# Autodesk Inventor assembly: Main_Station
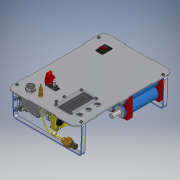
[picture p0: Inventor's stored thumbnail of the model, 180x180]
Saved by Autodesk Inventor 2016 (Build 200138000, 138)
## iProperties
Created: 2016-03-26
Part Number: Main_Station
Document SubType Name: Assembly
Designer: agmle
Author: agmle
## Documents named in this file (42)
- C:\Users\agmle\BitTorrent Sync\private\projects\Creekfleet_Timer\hardware\CAD\Main\Main_Station.iam
- C:\Users\agmle\BitTorrent Sync\private\projects\Creekfleet_Timer\hardware\CAD\Main\Case.ipt
- C:\Users\agmle\BitTorrent Sync\private\projects\Creekfleet_Timer\hardware\CAD\Main\Panel_Strut.ipt
- C:\Users\agmle\BitTorrent Sync\private\projects\Creekfleet_Timer\hardware\CAD\Main\VIAIR 90Cviair_90c_compressor_avp.ipt
- C:\Users\agmle\BitTorrent Sync\private\projects\Creekfleet_Timer\hardware\CAD\Main\Compressor_Strut.ipt
- C:\Users\agmle\BitTorrent Sync\private\projects\Creekfleet_Timer\hardware\CAD\Main\Panel.ipt
- C:\Users\agmle\BitTorrent Sync\private\projects\Creekfleet_Timer\hardware\CAD\Main\RKF 46-1M_NPT.ipt
- C:\Users\agmle\Documents\Inventor\Content Center Files\R2016\en-US\ANSI B18.22.1\ANSI B18.22.1 - No. 4 - Regular - Type B.ipt
- C:\Users\agmle\Documents\Inventor\Content Center Files\R2016\en-US\ANSI B18.22.1\ANSI B18.22.1 - 1_4 - narrow - Type B.ipt
- C:\Users\agmle\Documents\Inventor\Content Center Files\R2016\en-US\ASME B18.21.1(08)\ASME B18.21.1 - No. 4. Carbon Steel(2) A.ipt
- C:\Users\agmle\Documents\Inventor\Content Center Files\R2016\en-US\ASME B18.21.1(08)\ASME B18.21.1 - 1_4. Carbon Steel(2) A.ipt
- C:\Users\agmle\Documents\Inventor\Content Center Files\R2016\en-US\ANSI B18.3(03)\ANSI B18.3 - 1_4-20 UNC - UNC - 0.625(1).ipt
- C:\Users\agmle\Documents\Inventor\Content Center Files\R2016\en-US\ANSI B18.3(05)\ANSI B18.3 - 4-40 UNC - 0.3125(31).ipt
- C:\Users\agmle\BitTorrent Sync\private\projects\Creekfleet_Timer\hardware\CAD\Main\LCD.iam
- C:\Users\agmle\BitTorrent Sync\private\projects\Creekfleet_Timer\hardware\CAD\Main\LCD_Cover.ipt
- C:\Users\agmle\Documents\Inventor\Content Center Files\R2016\en-US\ANSI B18.3(05)\ANSI B18.3 - 4-40 UNC - 0.875(31).ipt
- C:\Users\agmle\Documents\Inventor\Content Center Files\R2016\en-US\ANSI B18.6.3(36)\ANSI B18.6.3 - 4 - 40(2).ipt
- C:\Users\agmle\BitTorrent Sync\private\projects\Creekfleet_Timer\hardware\CAD\Main\toggle switch cover.iam
- C:\Users\agmle\BitTorrent Sync\private\projects\Creekfleet_Timer\hardware\CAD\Main\Button_blue.iam
- C:\Users\agmle\BitTorrent Sync\private\projects\Creekfleet_Timer\hardware\CAD\Main\Button_green.iam
- C:\Users\agmle\BitTorrent Sync\private\projects\Creekfleet_Timer\hardware\CAD\Main\Button_red.iam
- C:\Users\agmle\BitTorrent Sync\private\projects\Creekfleet_Timer\hardware\CAD\Main\9414K930.ipt
- C:\Users\agmle\BitTorrent Sync\private\projects\Creekfleet_Timer\hardware\CAD\Main\9414K360.ipt
- C:\Users\agmle\BitTorrent Sync\private\projects\Creekfleet_Timer\hardware\CAD\Main\5454K650.ipt
- C:\Users\agmle\BitTorrent Sync\private\projects\Creekfleet_Timer\hardware\CAD\Main\50745K260.ipt
- C:\Users\agmle\BitTorrent Sync\private\projects\Creekfleet_Timer\hardware\CAD\Main\PX3AN2BS250PAAAX.ipt
- C:\Users\agmle\BitTorrent Sync\private\projects\Creekfleet_Timer\hardware\CAD\Main\2844K430.ipt
- C:\Users\agmle\BitTorrent Sync\private\projects\Creekfleet_Timer\hardware\CAD\Main\Main_Station\AIP\Tube and Pipe\Main_Station.Airline.iam
- C:\Users\agmle\BitTorrent Sync\private\projects\Creekfleet_Timer\hardware\CAD\Main\Toggle_Switch.iam
- C:\Users\agmle\BitTorrent Sync\private\projects\Creekfleet_Timer\hardware\CAD\Main\Toggle_Nut.ipt
- C:\Users\agmle\BitTorrent Sync\private\projects\Creekfleet_Timer\hardware\CAD\Main\BMS.ipt
- C:\Users\agmle\BitTorrent Sync\private\projects\Creekfleet_Timer\hardware\CAD\Main\40152S.ipt
- C:\Users\agmle\BitTorrent Sync\private\projects\Creekfleet_Timer\hardware\CAD\Main\Cell_Spacer.ipt
- C:\Users\agmle\BitTorrent Sync\private\projects\Creekfleet_Timer\hardware\CAD\Main\black_pp45.ipt
- C:\Users\agmle\BitTorrent Sync\private\projects\Creekfleet_Timer\hardware\CAD\Main\red_pp45.ipt
- C:\Users\agmle\BitTorrent Sync\private\projects\Creekfleet_Timer\hardware\CAD\Main\1470g1.ipt
- C:\Users\agmle\BitTorrent Sync\private\projects\Creekfleet_Timer\hardware\CAD\Main\AFB0512HA.ipt
- C:\Users\agmle\BitTorrent Sync\private\projects\Creekfleet_Timer\hardware\CAD\Main\Fan_Bracket.ipt
- C:\Users\agmle\Documents\Inventor\Content Center Files\R2016\en-US\ANSI B18.22.1\ANSI B18.22.1 - No. 8 - narrow - Type B.ipt
- C:\Users\agmle\Documents\Inventor\Content Center Files\R2016\en-US\ANSI B18.6.3(36)\ANSI B18.6.3 - 10 - 32(2).ipt
- C:\Users\agmle\Documents\Inventor\Content Center Files\R2016\en-US\ANSI B18.3(05)\ANSI B18.3 - 8-36 UNF - 0.875(31).ipt
- C:\Users\agmle\Documents\Inventor\Content Center Files\R2016\en-US\ASME B18.21.1(08)\ASME B18.21.1 - No. 8. Carbon Steel(2) A.ipt
## Components (123 placed, 41 different names)
1. Case:1 — Mate:1, Mate:2, Mate:3, Mate:4, Mate:5, Mate:6, Mate:7, Mate:8, Angle:2, Angle:3
2. Panel_Strut:1 — Mate:1, Mate:2, Mate:6, Insert:17, Insert:20, Insert:21, Mate:36, Mate:37, Mate:38, Angle:6
3. Panel_Strut:2 — Mate:3, Mate:4, Mate:5, Insert:14, Insert:16, Insert:22, Flush:2, Mate:35
4. VIAIR 90Cviair_90c_compressor_avp:1 — Insert:23, Insert:24, Insert:54, Insert:55, Insert:56, Insert:57, Insert:100
5. Compressor_Strut:1 — Insert:14, Insert:20, Insert:24, Insert:50, Insert:52, Mate:16
6. Compressor_Strut:2 — Insert:16, Insert:17, Insert:23, Insert:51, Insert:53
7. Panel:1 — Insert:21, Insert:22, Insert:25, Insert:46, Insert:47, Insert:48, Flush:1, Insert:74, Insert:87, Insert:88, Insert:94, Insert:95, Insert:96, Insert:97, Insert:98, Insert:102, Angle:5, Mate:17, Mate:34, Mate:41, Mate:42, Mate:43, Insert:125, Mate:49, Insert:130, Insert:131
8. RKF 46-1M_NPT:1 — Insert:25
9. Plain Washer (Inch) No. 4 - Regular - Type B:1 — Insert:30, Insert:46
10. Plain Washer (Inch) No. 4 - Regular - Type B:2 — Insert:31, Insert:47
11. Plain Washer (Inch) No. 4 - Regular - Type B:3 — Insert:32, Insert:48
12. Plain Washer (Inch) No. 4 - Regular - Type B:5 — Insert:34, Insert:50
13. Plain Washer (Inch) No. 4 - Regular - Type B:6 — Insert:35, Insert:51
14. Plain Washer (Inch) No. 4 - Regular - Type B:7 — Insert:36, Insert:52
15. Plain Washer (Inch) No. 4 - Regular - Type B:8 — Insert:37, Insert:53
16. Plain Washer (Inch) 1/4 - narrow - Type B:1 — Insert:29, Insert:56
17. Plain Washer (Inch) 1/4 - narrow - Type B:2 — Insert:28, Insert:57
18. Plain Washer (Inch) 1/4 - narrow - Type B:3 — Insert:27, Insert:55
19. Plain Washer (Inch) 1/4 - narrow - Type B:4 — Insert:26, Insert:54
20. Internal Tooth Lock Washer - Type A (Inch) No. 4. Carbon Steel:1 — Insert:30, Insert:45
21. Internal Tooth Lock Washer - Type A (Inch) No. 4. Carbon Steel:2 — Insert:31, Insert:44
22. Internal Tooth Lock Washer - Type A (Inch) No. 4. Carbon Steel:3 — Insert:32, Insert:43
23. Internal Tooth Lock Washer - Type A (Inch) No. 4. Carbon Steel:5 — Insert:34, Insert:41
24. Internal Tooth Lock Washer - Type A (Inch) No. 4. Carbon Steel:6 — Insert:35, Insert:40
25. Internal Tooth Lock Washer - Type A (Inch) No. 4. Carbon Steel:7 — Insert:36, Insert:39
26. Internal Tooth Lock Washer - Type A (Inch) No. 4. Carbon Steel:8 — Insert:37, Insert:38
27. Internal Tooth Lock Washer - Type A (Inch) 1/4. Carbon Steel:1 — Insert:26
28. Internal Tooth Lock Washer - Type A (Inch) 1/4. Carbon Steel:2 — Insert:27
29. Internal Tooth Lock Washer - Type A (Inch) 1/4. Carbon Steel:3 — Insert:28
30. Internal Tooth Lock Washer - Type A (Inch) 1/4. Carbon Steel:4 — Insert:29
31. Hexagon Socket Head Cap Screw - Inch No. 4 - 40 UNC - 5/16:2 — Insert:45
32. Hexagon Socket Head Cap Screw - Inch No. 4 - 40 UNC - 5/16:3 — Insert:44
33. Hexagon Socket Head Cap Screw - Inch No. 4 - 40 UNC - 5/16:4 — Insert:43
34. Hexagon Socket Head Cap Screw - Inch No. 4 - 40 UNC - 5/16:6 — Insert:41
35. Hexagon Socket Head Cap Screw - Inch No. 4 - 40 UNC - 5/16:7 — Insert:40
36. Hexagon Socket Head Cap Screw - Inch No. 4 - 40 UNC - 5/16:1 — Insert:39
37. Hexagon Socket Head Cap Screw - Inch No. 4 - 40 UNC - 5/16:8 — Insert:38
38. Hexagon Socket Button Head Cap Screw - Inch 1/4 - 20 x 5/8:1
39. Hexagon Socket Button Head Cap Screw - Inch 1/4 - 20 x 5/8:2
40. Hexagon Socket Button Head Cap Screw - Inch 1/4 - 20 x 5/8:3
41. Hexagon Socket Button Head Cap Screw - Inch 1/4 - 20 x 5/8:4
42. LCD:1 [sub-assembly] — Flush:1, Mate:9, Mate:10, Insert:79, Insert:80, Insert:81, Insert:82
43. LCD_Cover:1 — Insert:87, Insert:88, Insert:89, Insert:90, Insert:91, Insert:92
44. Plain Washer (Inch) No. 4 - Regular - Type B:9 — Insert:64, Insert:74
45. Plain Washer (Inch) No. 4 - Regular - Type B:10 — Insert:65, Insert:89
46. Plain Washer (Inch) No. 4 - Regular - Type B:11 — Insert:66, Insert:90
47. Plain Washer (Inch) No. 4 - Regular - Type B:12 — Insert:67, Insert:91
48. Plain Washer (Inch) No. 4 - Regular - Type B:13 — Insert:68, Insert:92
49. Internal Tooth Lock Washer - Type A (Inch) No. 4. Carbon Steel:9 — Insert:64, Insert:69
50. Internal Tooth Lock Washer - Type A (Inch) No. 4. Carbon Steel:10 — Insert:65, Insert:70
51. Internal Tooth Lock Washer - Type A (Inch) No. 4. Carbon Steel:11 — Insert:66, Insert:71
52. Internal Tooth Lock Washer - Type A (Inch) No. 4. Carbon Steel:12 — Insert:67, Insert:72
53. Internal Tooth Lock Washer - Type A (Inch) No. 4. Carbon Steel:13 — Insert:68, Insert:73
54. Hexagon Socket Head Cap Screw - Inch No. 4 - 40 UNC - 5/16:9 — Insert:69
55. Hexagon Socket Head Cap Screw - Inch No. 4 - 40 UNC - 7/8:2 — Insert:70, Mate:9
56. Hexagon Socket Head Cap Screw - Inch No. 4 - 40 UNC - 7/8:1 — Insert:71
57. Hexagon Socket Head Cap Screw - Inch No. 4 - 40 UNC - 7/8:3 — Insert:72, Mate:10
58. Hexagon Socket Head Cap Screw - Inch No. 4 - 40 UNC - 7/8:4 — Insert:73
59. Hex Machine Screw Nut - Inch 4 - 40:1 — Insert:79, Insert:86
60. Hex Machine Screw Nut - Inch 4 - 40:2 — Insert:80, Insert:83
61. Hex Machine Screw Nut - Inch 4 - 40:3 — Insert:81, Insert:85
62. Hex Machine Screw Nut - Inch 4 - 40:4 — Insert:82, Insert:84
63. Hex Machine Screw Nut - Inch 4 - 40:5 — Insert:84
64. Hex Machine Screw Nut - Inch 4 - 40:6 — Insert:83
65. Hex Machine Screw Nut - Inch 4 - 40:7 — Insert:86
66. Hex Machine Screw Nut - Inch 4 - 40:8 — Insert:85
67. toggle switch cover:1 [sub-assembly] — Insert:94, Angle:3, Insert:103
68. Button_red:1 [sub-assembly] — Insert:95
69. Button_blue:1 [sub-assembly] — Insert:97
70. Button_green:1 [sub-assembly] — Insert:96
71. 9414K930:1 — Insert:98, Angle:2, Insert:99
72. 9414K360:1 — Insert:99
73. 5454K650:1 — Insert:100
74. 50745K260:1 — Insert:101, Mate:38, Mate:39, Mate:40
75. PX3AN2BS250PAAAX:1 — Insert:101, Mate:36, Mate:37
76. 2844K430:1 — Mate:39, Angle:6, Mate:40
77. Main_Station.Airline:1 [sub-assembly]
78. Toggle_Switch:1 [sub-assembly] — Insert:102, Angle:5
79. Toggle_Nut:1 — Insert:103
80. BMS:1 — Mate:16, Flush:2, Mate:17, Flush:12
81. 40152S:1 — Mate:18, Mate:19, Flush:3
82. 40152S:2 — Mate:20, Mate:21, Flush:9
83. 40152S:3 — Mate:22, Mate:23, Flush:8, Flush:9
84. 40152S:4 — Mate:24, Mate:25, Flush:3, Flush:4
85. 40152S:5 — Mate:26, Mate:27, Flush:7, Flush:8
86. 40152S:6 — Mate:32, Mate:33, Flush:5, Flush:6, Flush:10, Flush:11
87. 40152S:7 — Mate:28, Mate:29, Flush:6, Flush:7
88. 40152S:8 — Mate:30, Mate:31, Flush:4, Flush:5
89. Cell_Spacer:1 — Mate:18, Mate:20, Mate:22, Mate:24, Mate:26, Mate:28, Mate:30, Mate:32, Flush:10, Mate:34, Flush:12, Mate:35
90. Cell_Spacer:2 — Mate:19, Mate:21, Mate:23, Mate:25, Mate:27, Mate:29, Mate:31, Mate:33, Flush:11
91. black_pp45:1 — Flush:13, Mate:44, Mate:47, Flush:16
92. black_pp45:2 — Flush:15, Mate:45, Mate:47, Flush:16, Flush:18, Flush:20
93. red_pp45:1 — Flush:13, Flush:14, Mate:44, Mate:46, Flush:17
94. red_pp45:2 — Flush:14, Flush:15, Mate:45, Mate:46, Flush:18, Flush:19
95. 1470g1:2 — Mate:41, Mate:42, Mate:43, Flush:17, Flush:19, Flush:20
96. AFB0512HA:1 — Insert:104, Mate:48, Insert:121, Insert:122, Insert:123, Insert:124
97. Fan_Bracket:1 — Insert:104, Mate:48, Insert:117, Insert:118, Insert:119, Insert:120, Insert:125, Mate:49
98. Hexagon Socket Head Cap Screw - Inch 8-36 UNF - 0.875:2 — Insert:105
99. Plain Washer (Inch) No. 8 - narrow - Type B:1 — Insert:105, Insert:117
100. Plain Washer (Inch) No. 8 - narrow - Type B:2 — Insert:121
101. Internal Tooth Lock Washer - Type A (Inch) No. 8. Carbon Steel:4
102. Hex Machine Screw Nut - Inch 10 - 32:1
103. Hexagon Socket Head Cap Screw - Inch 8-36 UNF - 0.875:3
104. Plain Washer (Inch) No. 8 - narrow - Type B:3 — Insert:119
105. Plain Washer (Inch) No. 8 - narrow - Type B:4 — Insert:124
106. Internal Tooth Lock Washer - Type A (Inch) No. 8. Carbon Steel:3
107. Hex Machine Screw Nut - Inch 10 - 32:2
108. Hexagon Socket Head Cap Screw - Inch 8-36 UNF - 0.875:4
109. Plain Washer (Inch) No. 8 - narrow - Type B:5 — Insert:120
110. Plain Washer (Inch) No. 8 - narrow - Type B:6 — Insert:123
111. Internal Tooth Lock Washer - Type A (Inch) No. 8. Carbon Steel:2
112. Hex Machine Screw Nut - Inch 10 - 32:3
113. Hexagon Socket Head Cap Screw - Inch 8-36 UNF - 0.875:1
114. Plain Washer (Inch) No. 8 - narrow - Type B:7 — Insert:118
115. Plain Washer (Inch) No. 8 - narrow - Type B:8 — Insert:122
116. Internal Tooth Lock Washer - Type A (Inch) No. 8. Carbon Steel:1
117. Hex Machine Screw Nut - Inch 10 - 32:4
118. Plain Washer (Inch) No. 4 - Regular - Type B:14 — Insert:130
119. Internal Tooth Lock Washer - Type A (Inch) No. 4. Carbon Steel:14
120. Hexagon Socket Head Cap Screw - Inch No. 4 - 40 UNC - 7/8:5
121. Plain Washer (Inch) No. 4 - Regular - Type B:15 — Insert:131
122. Internal Tooth Lock Washer - Type A (Inch) No. 4. Carbon Steel:15
123. Hexagon Socket Head Cap Screw - Inch No. 4 - 40 UNC - 7/8:6
## Relationships (173: Insert 105, Mate 44, Flush 20, Angle 4)
- Mate:1: Case:1 ↔ Panel_Strut:1
- Mate:2: Case:1 ↔ Panel_Strut:1
- Mate:3: Case:1 ↔ Panel_Strut:2
- Mate:4: Case:1 ↔ Panel_Strut:2
- Mate:5: Case:1 ↔ Panel_Strut:2
- Mate:6: Case:1 ↔ Panel_Strut:1
- Insert:14: Panel_Strut:2 ↔ Compressor_Strut:1
- Insert:16: Panel_Strut:2 ↔ Compressor_Strut:2
- Insert:17: Panel_Strut:1 ↔ Compressor_Strut:2
- Insert:20: Panel_Strut:1 ↔ Compressor_Strut:1
- Insert:21: Panel_Strut:1 ↔ Panel:1
- Insert:22: Panel_Strut:2 ↔ Panel:1
- Insert:23: VIAIR 90Cviair_90c_compressor_avp:1 ↔ Compressor_Strut:2
- Insert:24: VIAIR 90Cviair_90c_compressor_avp:1 ↔ Compressor_Strut:1
- Insert:25: Panel:1 ↔ RKF 46-1M_NPT:1
- Insert:26: Plain Washer (Inch) 1/4 - narrow - Type B:4 ↔ Internal Tooth Lock Washer - Type A (Inch) 1/4. Carbon Steel:1
- Insert:27: Plain Washer (Inch) 1/4 - narrow - Type B:3 ↔ Internal Tooth Lock Washer - Type A (Inch) 1/4. Carbon Steel:2
- Insert:28: Plain Washer (Inch) 1/4 - narrow - Type B:2 ↔ Internal Tooth Lock Washer - Type A (Inch) 1/4. Carbon Steel:3
- Insert:29: Plain Washer (Inch) 1/4 - narrow - Type B:1 ↔ Internal Tooth Lock Washer - Type A (Inch) 1/4. Carbon Steel:4
- Insert:30: Plain Washer (Inch) No. 4 - Regular - Type B:1 ↔ Internal Tooth Lock Washer - Type A (Inch) No. 4. Carbon Steel:1
- Insert:31: Plain Washer (Inch) No. 4 - Regular - Type B:2 ↔ Internal Tooth Lock Washer - Type A (Inch) No. 4. Carbon Steel:2
- Insert:32: Plain Washer (Inch) No. 4 - Regular - Type B:3 ↔ Internal Tooth Lock Washer - Type A (Inch) No. 4. Carbon Steel:3
- Insert:34: Plain Washer (Inch) No. 4 - Regular - Type B:5 ↔ Internal Tooth Lock Washer - Type A (Inch) No. 4. Carbon Steel:5
- Insert:35: Plain Washer (Inch) No. 4 - Regular - Type B:6 ↔ Internal Tooth Lock Washer - Type A (Inch) No. 4. Carbon Steel:6
- Insert:36: Plain Washer (Inch) No. 4 - Regular - Type B:7 ↔ Internal Tooth Lock Washer - Type A (Inch) No. 4. Carbon Steel:7
- Insert:37: Plain Washer (Inch) No. 4 - Regular - Type B:8 ↔ Internal Tooth Lock Washer - Type A (Inch) No. 4. Carbon Steel:8
- Insert:38: Internal Tooth Lock Washer - Type A (Inch) No. 4. Carbon Steel:8 ↔ Hexagon Socket Head Cap Screw - Inch No. 4 - 40 UNC - 5/16:8
- Insert:39: Internal Tooth Lock Washer - Type A (Inch) No. 4. Carbon Steel:7 ↔ Hexagon Socket Head Cap Screw - Inch No. 4 - 40 UNC - 5/16:1
- Insert:40: Internal Tooth Lock Washer - Type A (Inch) No. 4. Carbon Steel:6 ↔ Hexagon Socket Head Cap Screw - Inch No. 4 - 40 UNC - 5/16:7
- Insert:41: Internal Tooth Lock Washer - Type A (Inch) No. 4. Carbon Steel:5 ↔ Hexagon Socket Head Cap Screw - Inch No. 4 - 40 UNC - 5/16:6
- Insert:43: Internal Tooth Lock Washer - Type A (Inch) No. 4. Carbon Steel:3 ↔ Hexagon Socket Head Cap Screw - Inch No. 4 - 40 UNC - 5/16:4
- Insert:44: Internal Tooth Lock Washer - Type A (Inch) No. 4. Carbon Steel:2 ↔ Hexagon Socket Head Cap Screw - Inch No. 4 - 40 UNC - 5/16:3
- Insert:45: Internal Tooth Lock Washer - Type A (Inch) No. 4. Carbon Steel:1 ↔ Hexagon Socket Head Cap Screw - Inch No. 4 - 40 UNC - 5/16:2
- Insert:46: Panel:1 ↔ Plain Washer (Inch) No. 4 - Regular - Type B:1
- Insert:47: Panel:1 ↔ Plain Washer (Inch) No. 4 - Regular - Type B:2
- Insert:48: Panel:1 ↔ Plain Washer (Inch) No. 4 - Regular - Type B:3
- Insert:50: Compressor_Strut:1 ↔ Plain Washer (Inch) No. 4 - Regular - Type B:5
- Insert:51: Compressor_Strut:2 ↔ Plain Washer (Inch) No. 4 - Regular - Type B:6
- Insert:52: Compressor_Strut:1 ↔ Plain Washer (Inch) No. 4 - Regular - Type B:7
- Insert:53: Compressor_Strut:2 ↔ Plain Washer (Inch) No. 4 - Regular - Type B:8
- Insert:54: VIAIR 90Cviair_90c_compressor_avp:1 ↔ Plain Washer (Inch) 1/4 - narrow - Type B:4
- Insert:55: VIAIR 90Cviair_90c_compressor_avp:1 ↔ Plain Washer (Inch) 1/4 - narrow - Type B:3
- Insert:56: VIAIR 90Cviair_90c_compressor_avp:1 ↔ Plain Washer (Inch) 1/4 - narrow - Type B:1
- Insert:57: VIAIR 90Cviair_90c_compressor_avp:1 ↔ Plain Washer (Inch) 1/4 - narrow - Type B:2
- [Insert]: Internal Tooth Lock Washer - Type A (Inch) 1/4. Carbon Steel:4 ↔ Hexagon Socket Button Head Cap Screw - Inch 1/4 - 20 x 5/8:1
- [Insert]: Internal Tooth Lock Washer - Type A (Inch) 1/4. Carbon Steel:3 ↔ Hexagon Socket Button Head Cap Screw - Inch 1/4 - 20 x 5/8:2
- [Insert]: Internal Tooth Lock Washer - Type A (Inch) 1/4. Carbon Steel:1 ↔ Hexagon Socket Button Head Cap Screw - Inch 1/4 - 20 x 5/8:3
- [Insert]: Internal Tooth Lock Washer - Type A (Inch) 1/4. Carbon Steel:2 ↔ Hexagon Socket Button Head Cap Screw - Inch 1/4 - 20 x 5/8:4
- Flush:1: Panel:1 ↔ LCD:1
- Mate:7: Case:1
- Mate:8: Case:1
- Insert:64: Plain Washer (Inch) No. 4 - Regular - Type B:9 ↔ Internal Tooth Lock Washer - Type A (Inch) No. 4. Carbon Steel:9
- Insert:65: Plain Washer (Inch) No. 4 - Regular - Type B:10 ↔ Internal Tooth Lock Washer - Type A (Inch) No. 4. Carbon Steel:10
- Insert:66: Plain Washer (Inch) No. 4 - Regular - Type B:11 ↔ Internal Tooth Lock Washer - Type A (Inch) No. 4. Carbon Steel:11
- Insert:67: Plain Washer (Inch) No. 4 - Regular - Type B:12 ↔ Internal Tooth Lock Washer - Type A (Inch) No. 4. Carbon Steel:12
- Insert:68: Plain Washer (Inch) No. 4 - Regular - Type B:13 ↔ Internal Tooth Lock Washer - Type A (Inch) No. 4. Carbon Steel:13
- Insert:69: Internal Tooth Lock Washer - Type A (Inch) No. 4. Carbon Steel:9 ↔ Hexagon Socket Head Cap Screw - Inch No. 4 - 40 UNC - 5/16:9
- Insert:70: Internal Tooth Lock Washer - Type A (Inch) No. 4. Carbon Steel:10 ↔ Hexagon Socket Head Cap Screw - Inch No. 4 - 40 UNC - 7/8:2
- Insert:71: Internal Tooth Lock Washer - Type A (Inch) No. 4. Carbon Steel:11 ↔ Hexagon Socket Head Cap Screw - Inch No. 4 - 40 UNC - 7/8:1
- Insert:72: Internal Tooth Lock Washer - Type A (Inch) No. 4. Carbon Steel:12 ↔ Hexagon Socket Head Cap Screw - Inch No. 4 - 40 UNC - 7/8:3
- Insert:73: Internal Tooth Lock Washer - Type A (Inch) No. 4. Carbon Steel:13 ↔ Hexagon Socket Head Cap Screw - Inch No. 4 - 40 UNC - 7/8:4
- Insert:74: Panel:1 ↔ Plain Washer (Inch) No. 4 - Regular - Type B:9
- Mate:9: LCD:1 ↔ Hexagon Socket Head Cap Screw - Inch No. 4 - 40 UNC - 7/8:2
- Mate:10: LCD:1 ↔ Hexagon Socket Head Cap Screw - Inch No. 4 - 40 UNC - 7/8:3
- Insert:79: LCD:1 ↔ Hex Machine Screw Nut - Inch 4 - 40:1
- Insert:80: LCD:1 ↔ Hex Machine Screw Nut - Inch 4 - 40:2
- Insert:81: LCD:1 ↔ Hex Machine Screw Nut - Inch 4 - 40:3
- Insert:82: LCD:1 ↔ Hex Machine Screw Nut - Inch 4 - 40:4
- Insert:83: Hex Machine Screw Nut - Inch 4 - 40:2 ↔ Hex Machine Screw Nut - Inch 4 - 40:6
- Insert:84: Hex Machine Screw Nut - Inch 4 - 40:4 ↔ Hex Machine Screw Nut - Inch 4 - 40:5
- Insert:85: Hex Machine Screw Nut - Inch 4 - 40:3 ↔ Hex Machine Screw Nut - Inch 4 - 40:8
- Insert:86: Hex Machine Screw Nut - Inch 4 - 40:1 ↔ Hex Machine Screw Nut - Inch 4 - 40:7
- Insert:87: Panel:1 ↔ LCD_Cover:1
- Insert:88: Panel:1 ↔ LCD_Cover:1
- Insert:89: LCD_Cover:1 ↔ Plain Washer (Inch) No. 4 - Regular - Type B:10
- Insert:90: LCD_Cover:1 ↔ Plain Washer (Inch) No. 4 - Regular - Type B:11
- Insert:91: LCD_Cover:1 ↔ Plain Washer (Inch) No. 4 - Regular - Type B:12
- Insert:92: LCD_Cover:1 ↔ Plain Washer (Inch) No. 4 - Regular - Type B:13
- Insert:94: Panel:1 ↔ toggle switch cover:1
- Insert:95: Panel:1 ↔ Button_red:1
- Insert:96: Panel:1 ↔ Button_green:1
- Insert:97: Panel:1 ↔ Button_blue:1
- Insert:98: Panel:1 ↔ 9414K930:1
- Angle:2 (0 deg): Case:1 ↔ 9414K930:1
- Angle:3 (180 deg): Case:1 ↔ toggle switch cover:1
- Insert:99: 9414K930:1 ↔ 9414K360:1
- Insert:100: VIAIR 90Cviair_90c_compressor_avp:1 ↔ 5454K650:1
- Insert:101: 50745K260:1 ↔ PX3AN2BS250PAAAX:1
- Insert:102: Panel:1 ↔ Toggle_Switch:1
- Insert:103: toggle switch cover:1 ↔ Toggle_Nut:1
- Angle:5 (0 deg): Panel:1 ↔ Toggle_Switch:1
- Mate:16: Compressor_Strut:1 ↔ BMS:1
- Flush:2 (25.4 mm): Panel_Strut:2 ↔ BMS:1
- Mate:17 (12.7 mm): Panel:1 ↔ BMS:1
- Mate:18: 40152S:1 ↔ Cell_Spacer:1
- Mate:19: 40152S:1 ↔ Cell_Spacer:2
- Mate:20: 40152S:2 ↔ Cell_Spacer:1
- Mate:21: 40152S:2 ↔ Cell_Spacer:2
- Mate:22: 40152S:3 ↔ Cell_Spacer:1
- Mate:23: 40152S:3 ↔ Cell_Spacer:2
- Mate:24: 40152S:4 ↔ Cell_Spacer:1
- Mate:25: 40152S:4 ↔ Cell_Spacer:2
- Mate:26: 40152S:5 ↔ Cell_Spacer:1
- Mate:27: 40152S:5 ↔ Cell_Spacer:2
- Mate:28: 40152S:7 ↔ Cell_Spacer:1
- Mate:29: 40152S:7 ↔ Cell_Spacer:2
- Mate:30: 40152S:8 ↔ Cell_Spacer:1
- Mate:31: 40152S:8 ↔ Cell_Spacer:2
- Mate:32: 40152S:6 ↔ Cell_Spacer:1
- Mate:33: 40152S:6 ↔ Cell_Spacer:2
- Flush:3: 40152S:1 ↔ 40152S:4
- Flush:4: 40152S:4 ↔ 40152S:8
- Flush:5: 40152S:6 ↔ 40152S:8
- Flush:6: 40152S:6 ↔ 40152S:7
- Flush:7: 40152S:5 ↔ 40152S:7
- Flush:8: 40152S:3 ↔ 40152S:5
- Flush:9: 40152S:2 ↔ 40152S:3
- Flush:10 (6.35 mm): 40152S:6 ↔ Cell_Spacer:1
- Flush:11 (6.35 mm): 40152S:6 ↔ Cell_Spacer:2
- Mate:34: Panel:1 ↔ Cell_Spacer:1
- Flush:12 (-31.75 mm): BMS:1 ↔ Cell_Spacer:1
- Mate:35 (12.7 mm): Panel_Strut:2 ↔ Cell_Spacer:1
- Mate:36: Panel_Strut:1 ↔ PX3AN2BS250PAAAX:1
- Mate:37: Panel_Strut:1 ↔ PX3AN2BS250PAAAX:1
- Mate:38 (177.8 mm): Panel_Strut:1 ↔ 50745K260:1
- Mate:39: 50745K260:1 ↔ 2844K430:1
- Angle:6 (160 deg): Panel_Strut:1 ↔ 2844K430:1
- Mate:40 (12.7 mm): 50745K260:1 ↔ 2844K430:1
- Mate:41: Panel:1 ↔ 1470g1:2
- Mate:42: Panel:1 ↔ 1470g1:2
- Mate:43: Panel:1 ↔ 1470g1:2
- Flush:13: black_pp45:1 ↔ red_pp45:1
- Flush:14: red_pp45:1 ↔ red_pp45:2
- Flush:15: black_pp45:2 ↔ red_pp45:2
- Mate:44: black_pp45:1 ↔ red_pp45:1
- Mate:45: black_pp45:2 ↔ red_pp45:2
- Mate:46: red_pp45:1 ↔ red_pp45:2
- Mate:47: black_pp45:1 ↔ black_pp45:2
- Flush:16: black_pp45:1 ↔ black_pp45:2
- Flush:17 (-3.175 mm): red_pp45:1 ↔ 1470g1:2
- Flush:18: black_pp45:2 ↔ red_pp45:2
- Flush:19 (3.175 mm): red_pp45:2 ↔ 1470g1:2
- Flush:20 (3.175 mm): black_pp45:2 ↔ 1470g1:2
- Insert:104: AFB0512HA:1 ↔ Fan_Bracket:1
- Mate:48: AFB0512HA:1 ↔ Fan_Bracket:1
- Insert:105: Hexagon Socket Head Cap Screw - Inch 8-36 UNF - 0.875:2 ↔ Plain Washer (Inch) No. 8 - narrow - Type B:1
- [Insert]: Internal Tooth Lock Washer - Type A (Inch) No. 8. Carbon Steel:4 ↔ Hex Machine Screw Nut - Inch 10 - 32:1
- [Insert]: Plain Washer (Inch) No. 8 - narrow - Type B:2 ↔ Internal Tooth Lock Washer - Type A (Inch) No. 8. Carbon Steel:4
- [Insert]: Hexagon Socket Head Cap Screw - Inch 8-36 UNF - 0.875:3 ↔ Plain Washer (Inch) No. 8 - narrow - Type B:3
- [Insert]: Internal Tooth Lock Washer - Type A (Inch) No. 8. Carbon Steel:3 ↔ Hex Machine Screw Nut - Inch 10 - 32:2
- [Insert]: Plain Washer (Inch) No. 8 - narrow - Type B:4 ↔ Internal Tooth Lock Washer - Type A (Inch) No. 8. Carbon Steel:3
- [Insert]: Hexagon Socket Head Cap Screw - Inch 8-36 UNF - 0.875:4 ↔ Plain Washer (Inch) No. 8 - narrow - Type B:5
- [Insert]: Internal Tooth Lock Washer - Type A (Inch) No. 8. Carbon Steel:2 ↔ Hex Machine Screw Nut - Inch 10 - 32:3
- [Insert]: Plain Washer (Inch) No. 8 - narrow - Type B:6 ↔ Internal Tooth Lock Washer - Type A (Inch) No. 8. Carbon Steel:2
- [Insert]: Hexagon Socket Head Cap Screw - Inch 8-36 UNF - 0.875:1 ↔ Plain Washer (Inch) No. 8 - narrow - Type B:7
- [Insert]: Internal Tooth Lock Washer - Type A (Inch) No. 8. Carbon Steel:1 ↔ Hex Machine Screw Nut - Inch 10 - 32:4
- [Insert]: Plain Washer (Inch) No. 8 - narrow - Type B:8 ↔ Internal Tooth Lock Washer - Type A (Inch) No. 8. Carbon Steel:1
- Insert:117: Fan_Bracket:1 ↔ Plain Washer (Inch) No. 8 - narrow - Type B:1
- Insert:118: Fan_Bracket:1 ↔ Plain Washer (Inch) No. 8 - narrow - Type B:7
- Insert:119: Fan_Bracket:1 ↔ Plain Washer (Inch) No. 8 - narrow - Type B:3
- Insert:120: Fan_Bracket:1 ↔ Plain Washer (Inch) No. 8 - narrow - Type B:5
- Insert:121: AFB0512HA:1 ↔ Plain Washer (Inch) No. 8 - narrow - Type B:2
- Insert:122: AFB0512HA:1 ↔ Plain Washer (Inch) No. 8 - narrow - Type B:8
- Insert:123: AFB0512HA:1 ↔ Plain Washer (Inch) No. 8 - narrow - Type B:6
- Insert:124: AFB0512HA:1 ↔ Plain Washer (Inch) No. 8 - narrow - Type B:4
- Insert:125: Panel:1 ↔ Fan_Bracket:1
- Mate:49: Panel:1 ↔ Fan_Bracket:1
- [Insert]: Plain Washer (Inch) No. 4 - Regular - Type B:14 ↔ Internal Tooth Lock Washer - Type A (Inch) No. 4. Carbon Steel:14
- [Insert]: Internal Tooth Lock Washer - Type A (Inch) No. 4. Carbon Steel:14 ↔ Hexagon Socket Head Cap Screw - Inch No. 4 - 40 UNC - 7/8:5
- [Insert]: Plain Washer (Inch) No. 4 - Regular - Type B:15 ↔ Internal Tooth Lock Washer - Type A (Inch) No. 4. Carbon Steel:15
- [Insert]: Internal Tooth Lock Washer - Type A (Inch) No. 4. Carbon Steel:15 ↔ Hexagon Socket Head Cap Screw - Inch No. 4 - 40 UNC - 7/8:6
- Insert:130: Panel:1 ↔ Plain Washer (Inch) No. 4 - Regular - Type B:14
- Insert:131: Panel:1 ↔ Plain Washer (Inch) No. 4 - Regular - Type B:15
## Named parameters: d196_d193 = 0 mm, d197_d194 = 0 mm, d198_d195 = 0 mm, d199_d193 = 0 mm, d200_d194 = 0 mm, d201_d195 = 0 mm, d202_d193 = 0 mm, d203_d194 = 0 mm, d204_d195 = 0 mm, d215_d85 = 0 mm, d216_d80 = 0 mm, d217_d85 = 0 mm, d218_d80 = 0 mm
